# Autodesk Inventor assembly: ASY ДМФ 070 кольцо под шпильки КОРМА наружное v2.0
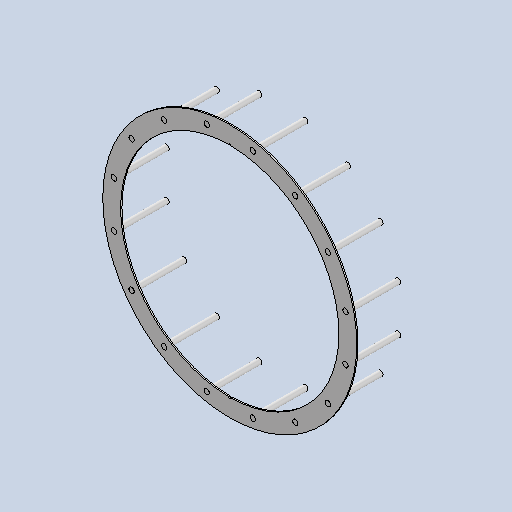
[picture p0: Inventor's stored thumbnail of the model, 512x512]
Saved by Autodesk Inventor 2025 (Build 290162010, 162A)
## iProperties
Created: 2024-05-08
Part Number: ASY ДМФ 070 кольцо под шпильки КОРМА наружное v2.0
Document SubType Name: Assembly
Designer: pokla
Stock Number: ДМФ 040 кольцо под шпильки КОРМА
Author: pokla
## Documents named in this file (4)
- C:\Users\admin\Yandex.Disk\home pc\Inventor\DMF-Disk-Micro-Filter\ASY ДМФ 070 кольцо под шпильки КОРМА наружное v2.0.iam
- C:\Users\admin\Yandex.Disk\home pc\Inventor\DMF-Disk-Micro-Filter\ДМФ 041 кольцо под шпильки КОРМА v2.0.ipt
- C:\Users\admin\Yandex.Disk\home pc\Inventor\DMF-Disk-Micro-Filter\ДМФ 042 шпилька 1 v2.0.ipt
- C:\Users\admin\Yandex.Disk\home pc\Inventor\DMF-Disk-Micro-Filter\ДМФ 000 размеры v2.0.ipt
## Components (17 placed, 2 different names)
1. ДМФ 041 кольцо под шпильки КОРМА v2.0.ipt:1 — Rigid:1
2. ДМФ 042 шпилька 1 v2.0.ipt:1 — Rigid:1
3. ДМФ 042 шпилька 1 v2.0.ipt:2
4. ДМФ 042 шпилька 1 v2.0.ipt:3
5. ДМФ 042 шпилька 1 v2.0.ipt:4
6. ДМФ 042 шпилька 1 v2.0.ipt:5
7. ДМФ 042 шпилька 1 v2.0.ipt:6
8. ДМФ 042 шпилька 1 v2.0.ipt:7
9. ДМФ 042 шпилька 1 v2.0.ipt:8
10. ДМФ 042 шпилька 1 v2.0.ipt:9
11. ДМФ 042 шпилька 1 v2.0.ipt:10
12. ДМФ 042 шпилька 1 v2.0.ipt:11
13. ДМФ 042 шпилька 1 v2.0.ipt:12
14. ДМФ 042 шпилька 1 v2.0.ipt:13
15. ДМФ 042 шпилька 1 v2.0.ipt:14
16. ДМФ 042 шпилька 1 v2.0.ipt:15
17. ДМФ 042 шпилька 1 v2.0.ipt:16
## Component patterns: (16 elements, first: ДМФ 042 шпилька 1 v2.0.ipt:1)
## Relationships (1: WeldJoint 1)
- Rigid:1 [WeldJoint]: ДМФ 041 кольцо под шпильки КОРМА v2.0.ipt:1 ↔ ДМФ 042 шпилька 1 v2.0.ipt:1
